# Autodesk Inventor assembly: Battery Tube
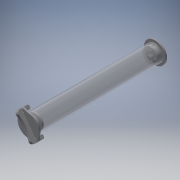
[picture p0: Inventor's stored thumbnail of the model, 180x180]
Saved by Autodesk Inventor 2016 (Build 200138000, 138)
## iProperties
Created: 2015-06-17
Part Number: Battery Tube
Document SubType Name: Assembly
Designer: JR
Author: JR
## Documents named in this file (11)
- D:\OpenROV\2.8\Github Official\Inventor\Battery Tubes\Battery Tube.iam
- D:\OpenROV\2.8\Github Official\Inventor\Battery Tubes\Aft\Aft Endcap Inner.ipt
- D:\OpenROV\2.8\Github Official\Inventor\Battery Tubes\Aft\Aft Endcap Middle.ipt
- D:\OpenROV\2.8\Github Official\Inventor\Battery Tubes\Aft\Aft Endcap Outer.ipt
- D:\OpenROV\2.8\Github Official\Inventor\Battery Tubes\Forward\Battery Tube Collar.ipt
- D:\OpenROV\2.8\Github Official\Inventor\Battery Tubes\BatteryTube.ipt
- D:\OpenROV\2.8\Github Official\Inventor\Battery Tubes\Forward\Forward Endcap 3mm.ipt
- D:\OpenROV\2.8\Github Official\Inventor\Battery Tubes\Forward\ForwardEndcap_6millimeter.ipt
- D:\OpenROV\2.8\Github Official\Inventor\Battery Tubes\Forward\FrontTerm.ipt
- D:\OpenROV\2.8\Github Official\Inventor\Battery Tubes\Forward\Twist Lock.ipt
- D:\OpenROV\2.8\Github Official\Inventor\Battery Tubes\Forward\Forward Endcap Outer.ipt
## Components (11 placed, 10 different names)
1. BatteryTube:1 — Mate:3, Flush:3, Insert:6, Insert:7, Mate:4
2. Aft Endcap Inner:1 — Insert:5
3. Aft Endcap Middle:1 — Insert:4, Flush:1, Insert:5
4. Aft Endcap Outer:1 — Insert:4, Flush:1, Insert:7
5. Battery Tube Collar:1 — Mate:3, Flush:3
6. Forward Endcap 3mm:1 — Insert:3
7. Forward Endcap 3mm:2 — Insert:1, Insert:2
8. ForwardEndcap_6millimeter:1 — Insert:2, Insert:3
9. FrontTerm:1 — Mate:4
10. Twist Lock:1 — Mate:1, Mate:2, Flush:2
11. Forward Endcap Outer:1 — Insert:1, Mate:1, Mate:2, Flush:2, Insert:6
## Relationships (14: Insert 7, Mate 4, Flush 3)
- Insert:1: Forward Endcap 3mm:2 ↔ Forward Endcap Outer:1
- Insert:2: Forward Endcap 3mm:2 ↔ ForwardEndcap_6millimeter:1
- Insert:3: Forward Endcap 3mm:1 ↔ ForwardEndcap_6millimeter:1
- Insert:4: Aft Endcap Middle:1 ↔ Aft Endcap Outer:1
- Flush:1: Aft Endcap Middle:1 ↔ Aft Endcap Outer:1
- Insert:5: Aft Endcap Inner:1 ↔ Aft Endcap Middle:1
- Mate:1: Twist Lock:1 ↔ Forward Endcap Outer:1
- Mate:2: Twist Lock:1 ↔ Forward Endcap Outer:1
- Flush:2: Twist Lock:1 ↔ Forward Endcap Outer:1
- Mate:3: BatteryTube:1 ↔ Battery Tube Collar:1
- Flush:3: BatteryTube:1 ↔ Battery Tube Collar:1
- Insert:6: BatteryTube:1 ↔ Forward Endcap Outer:1
- Insert:7: BatteryTube:1 ↔ Aft Endcap Outer:1
- Mate:4: BatteryTube:1 ↔ FrontTerm:1
